# Autodesk Inventor assembly: flop down intake part
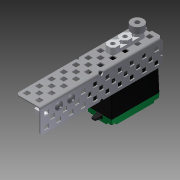
[picture p0: Inventor's stored thumbnail of the model, 180x180]
Saved by Autodesk Inventor 2014 (Build 180170000, 170)
## iProperties
Created: 2013-09-20
Part Number: flop down intake part
Document SubType Name: Assembly
Designer: Ryan
Author: Ryan
## Documents named in this file (8)
- C:\Users\Ryan\Desktop\sw\toss up robot intake\flop down intake part.iam
- C:\Users\Ryan\Desktop\sw\lib\Aperture VEX CAD Library\Bearing Blocks\Bearing Block.ipt
- C:\Users\Ryan\Desktop\sw\lib\Aperture VEX CAD Library\Metal\L Bar\2 x 10.ipt
- C:\Users\Ryan\Desktop\sw\lib\Aperture VEX CAD Library\Hardware\8-32\8-32_.500.ipt
- C:\Users\Ryan\Desktop\sw\lib\Aperture VEX CAD Library\Hardware\8-32\locknut (copy).ipt
- C:\Users\Ryan\Desktop\sw\lib\Super Sonic Sparks VEX CAD Library\Motors & Sensors\2-Wire Motor 393-Without Wire.iam
- C:\Users\Ryan\Desktop\sw\lib\Aperture VEX CAD Library\Spacers\SPACER-0500-0250.ipt
- C:\Users\Ryan\Desktop\sw\lib\Aperture VEX CAD Library\Hardware\Shaft Collar.ipt
## Components (11 placed, 7 different names)
1. Bearing Block:1 — Mate:1, Mate:2, Mate:3, Mate:4, Mate:5, Mate:9, Mate:10, Mate:13
2. 2 x 10:1 — Mate:1, Mate:2, Mate:3, Mate:4, Mate:6, Mate:8, Mate:14, Mate:15, Mate:16, Mate:17, Mate:18, Mate:23
3. 8-32_.500:1 — Mate:5, Mate:6, Mate:11
4. 8-32_.500:2 — Mate:8, Mate:9, Mate:12
5. locknut (copy):1 — Mate:10, Mate:11
6. locknut (copy):2 — Mate:12, Mate:13
7. 2-Wire Motor 393-Without Wire:1 [sub-assembly] — Mate:14, Mate:19, Mate:20, Mate:21
8. Bearing Block:2 — Mate:15, Mate:16, Mate:17, Mate:18, Mate:19, Mate:20, Mate:22, Mate:24, Mate:25, Mate:26
9. SPACER-0500-0250:1 — Mate:23, Mate:24
10. Shaft Collar:1 — Mate:21, Mate:22
11. SPACER-0500-0250:2 — Mate:25, Mate:26
## Relationships (25: Mate 25)
- Mate:1: Bearing Block:1 ↔ 2 x 10:1
- Mate:2 (2.3114 mm): Bearing Block:1 ↔ 2 x 10:1
- Mate:3 (2.3114 mm): Bearing Block:1 ↔ 2 x 10:1
- Mate:4 (2.3114 mm): Bearing Block:1 ↔ 2 x 10:1
- Mate:5: Bearing Block:1 ↔ 8-32_.500:1
- Mate:6: 2 x 10:1 ↔ 8-32_.500:1
- Mate:8: 2 x 10:1 ↔ 8-32_.500:2
- Mate:9: Bearing Block:1 ↔ 8-32_.500:2
- Mate:10: Bearing Block:1 ↔ locknut (copy):1
- Mate:11: 8-32_.500:1 ↔ locknut (copy):1
- Mate:12: 8-32_.500:2 ↔ locknut (copy):2
- Mate:13: Bearing Block:1 ↔ locknut (copy):2
- Mate:14: 2 x 10:1 ↔ 2-Wire Motor 393-Without Wire:1
- Mate:15: 2 x 10:1 ↔ Bearing Block:2
- Mate:16 (2.3114 mm): 2 x 10:1 ↔ Bearing Block:2
- Mate:17 (2.3114 mm): 2 x 10:1 ↔ Bearing Block:2
- Mate:18 (2.3114 mm): 2 x 10:1 ↔ Bearing Block:2
- Mate:19: 2-Wire Motor 393-Without Wire:1 ↔ Bearing Block:2
- Mate:20: 2-Wire Motor 393-Without Wire:1 ↔ Bearing Block:2
- Mate:21: 2-Wire Motor 393-Without Wire:1 ↔ Shaft Collar:1
- Mate:22: Bearing Block:2 ↔ Shaft Collar:1
- Mate:23: 2 x 10:1 ↔ SPACER-0500-0250:1
- Mate:24: Bearing Block:2 ↔ SPACER-0500-0250:1
- Mate:25: Bearing Block:2 ↔ SPACER-0500-0250:2
- Mate:26: Bearing Block:2 ↔ SPACER-0500-0250:2
## Named parameters: q = 2.3114 mm
